# Autodesk Inventor assembly: alpha
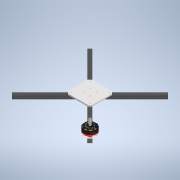
[picture p0: Inventor's stored thumbnail of the model, 180x180]
Saved by Autodesk Inventor 2021 (Build 250183000, 183)
## iProperties
Created: 2020-04-12
Part Number: alpha
Document SubType Name: Assembly
Designer: chutsu
Author: chutsu
## Documents named in this file (5)
- C:\Users\chutsu\Documents\alpha\alpha.iam
- C:\Users\chutsu\Documents\alpha\Top Plate.ipt
- C:\Users\chutsu\Documents\alpha\Carbon Fiber Arm.ipt
- C:\Users\chutsu\Documents\alpha\Motor Mount.ipt
- C:\Users\chutsu\Documents\alpha\EMAX RS2205 S\EMAX RS2205S.iam
## Components (7 placed, 4 different names)
1. Top Plate:1 — Rotational:1, Rotational:2, Rotational:3, Rotational:4, Rotational:5, Rotational:6, Rotational:7, Rotational:8
2. Carbon Fiber Arm:1 — Rotational:1, Rotational:2
3. Carbon Fiber Arm:2 — Rotational:3, Rotational:4
4. Carbon Fiber Arm:3 — Rotational:5, Rotational:6
5. Carbon Fiber Arm:4 — Rotational:7, Rotational:8, Mate:1, Mate:2
6. EMAX RS2205S:1 [sub-assembly] — Mate:3
7. Motor Mount:1 — Mate:1, Mate:2, Mate:3
## Relationships (11: RevoluteJoint 8, Mate 3)
- Rotational:1 [RevoluteJoint]: Top Plate:1 ↔ Carbon Fiber Arm:1
- Rotational:2 [RevoluteJoint]: Top Plate:1 ↔ Carbon Fiber Arm:1
- Rotational:3 [RevoluteJoint]: Top Plate:1 ↔ Carbon Fiber Arm:2
- Rotational:4 [RevoluteJoint]: Top Plate:1 ↔ Carbon Fiber Arm:2
- Rotational:5 [RevoluteJoint]: Top Plate:1 ↔ Carbon Fiber Arm:3
- Rotational:6 [RevoluteJoint]: Top Plate:1 ↔ Carbon Fiber Arm:3
- Rotational:7 [RevoluteJoint]: Top Plate:1 ↔ Carbon Fiber Arm:4
- Rotational:8 [RevoluteJoint]: Top Plate:1 ↔ Carbon Fiber Arm:4
- Mate:1: Carbon Fiber Arm:4 ↔ Motor Mount:1
- Mate:2: Carbon Fiber Arm:4 ↔ Motor Mount:1
- Mate:3: EMAX RS2205S:1 ↔ Motor Mount:1
